# Autodesk Inventor assembly: reducer_leg
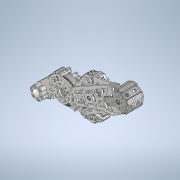
[picture p0: Inventor's stored thumbnail of the model, 180x180]
Saved by Autodesk Inventor 2020 (Build 240168000, 168)
## iProperties
Created: 2020-07-04
Part Number: reducer_leg
Document SubType Name: Assembly
Designer: psrobotics
Author: psrobotics
## Documents named in this file (26)
- D:\projects-3\biped_gen1\hardware\reducer_leg.iam
- D:\projects-3\biped_gen1\hardware\90_motor.iam
- D:\projects-3\biped_gen1\hardware\xl_20.ipt
- D:\projects-3\biped_gen1\hardware\xl_wheel_ass.iam
- D:\projects-3\biped_gen1\hardware\shell_2.ipt
- D:\projects-3\biped_gen1\hardware\shell_3.ipt
- D:\projects-3\biped_gen1\hardware\shell_4.ipt
- D:\projects-3\biped_gen1\hardware\motor_h_1.ipt
- D:\projects-3\biped_gen1\hardware\shell_5.ipt
- D:\projects-3\biped_gen1\hardware\bearing_shell_1.ipt
- D:\projects-3\biped_gen1\hardware\bearing_shell_2.ipt
- D:\projects-3\biped_gen1\hardware\xl_30_1.ipt
- D:\projects-3\biped_gen1\hardware\motor_h_4.ipt
- D:\projects-3\biped_gen1\hardware\motor_h_3_m.ipt
- D:\projects-3\biped_gen1\hardware\motor_h_5_m.ipt
- D:\projects-3\biped_gen1\hardware\bearing_35_44_5.ipt
- D:\projects-3\biped_gen1\hardware\motor_r_1.ipt
- D:\projects-3\biped_gen1\hardware\bearing_8_16_5.ipt
- D:\projects-3\biped_gen1\hardware\bearing_6_13_5.ipt
- D:\projects-3\biped_gen1\hardware\bearing_shell_3.ipt
- D:\projects-3\biped_gen1\hardware\joint_connector_1.ipt
- D:\projects-3\biped_gen1\hardware\joint_connector_2.ipt
- D:\projects-3\biped_gen1\hardware\end_holder_2.ipt
- D:\projects-3\biped_gen1\hardware\motor_h_6.ipt
- D:\projects-3\biped_gen1\hardware\end_holder_3.ipt
- D:\projects-3\biped_gen1\hardware\end_holder_4.ipt
## Components (33 placed, 25 different names)
1. 90_motor:1 [sub-assembly] — Insert:1, Insert:2, Flush:4, Insert:58, Insert:59
2. xl_20:1 — Insert:1, Insert:2, Flush:1, Tangent:1
3. xl_wheel_ass:1 [sub-assembly] — Flush:1, Tangent:1, Insert:9
4. shell_2:1 — Angle:1, Insert:9, Insert:18
5. shell_2:3 — Angle:1, Angle:2, Insert:14, Insert:17
6. shell_2:4 — Angle:2, Flush:6, Insert:15, Insert:16, Insert:33, Insert:34, Insert:81, Insert:82
7. shell_3:1 — Flush:4, Flush:5, Insert:25, Insert:26, Insert:42, Insert:43
8. shell_4:1 — Flush:5, Insert:25, Insert:26, Flush:12, Insert:40, Insert:41
9. motor_h_1:1 — Flush:6, Insert:14, Insert:15, Insert:16, Insert:17, Insert:18, Flush:10, Insert:27, Insert:28, Insert:30, Insert:31, Insert:52, Insert:53
10. shell_5:1 — Insert:35, Insert:36, Insert:37, Insert:38
11. bearing_shell_2:1 — Flush:10, Insert:27, Insert:28, Insert:75
12. xl_wheel_ass:2 [sub-assembly] — Insert:32
13. xl_30_1:1 — Insert:89
14. bearing_shell_1:1 — Insert:30, Insert:31, Insert:32
15. motor_h_4:1 — Insert:33, Insert:34, Insert:37, Insert:38, Insert:54, Insert:78, Insert:79, Flush:21, Flush:22, Flush:23, Insert:85, Insert:86, Insert:87
16. motor_h_3_m:1 — Insert:35, Insert:36, Insert:42, Insert:43, Flush:15, Insert:47, Insert:48, Insert:58, Insert:59, Flush:18, Insert:63, Insert:64, Flush:19, Insert:65, Insert:66
17. motor_h_5_m:1 — Flush:12, Insert:40, Insert:41
18. bearing_35_44_5:1 — Insert:77, Insert:87
19. motor_r_1:1 — Flush:15, Insert:47, Insert:48, Flush:17, Insert:60, Insert:61, Flush:24
20. bearing_8_16_5:1 — Insert:88, Insert:89
21. bearing_8_16_5:2 — Insert:52
22. bearing_8_16_5:3 — Insert:54
23. bearing_8_16_5:4 — Insert:53
24. bearing_6_13_5:1 — Insert:75
25. bearing_shell_3:1 — Flush:17, Insert:60, Insert:61, Insert:76
26. bearing_8_16_5:5 — Insert:76
27. joint_connector_1:1 — Flush:18, Insert:63, Insert:64
28. joint_connector_2:1 — Flush:19, Insert:65, Insert:66
29. bearing_35_44_5:2 — Insert:77, Flush:20
30. end_holder_2:1 — Insert:78, Insert:79, Flush:24, Insert:88
31. motor_h_6:1 — Flush:20, Insert:81, Insert:82, Insert:83, Insert:84
32. end_holder_3:1 — Flush:21, Flush:22, Insert:83, Insert:84
33. end_holder_4:1 — Flush:23, Insert:85, Insert:86
## Relationships (70: Insert 52, Flush 15, Angle 2, Tangent 1)
- Insert:1: 90_motor:1 ↔ xl_20:1
- Insert:2: 90_motor:1 ↔ xl_20:1
- Flush:1: xl_20:1 ↔ xl_wheel_ass:1
- Tangent:1 (1.3 mm): xl_20:1 ↔ xl_wheel_ass:1
- Angle:1 (160 deg): shell_2:1 ↔ shell_2:3
- Angle:2 (230 deg): shell_2:3 ↔ shell_2:4
- Insert:9 (-0.5 mm): xl_wheel_ass:1 ↔ shell_2:1
- Flush:4: 90_motor:1 ↔ shell_3:1
- Flush:5: shell_3:1 ↔ shell_4:1
- Flush:6: shell_2:4 ↔ motor_h_1:1
- Insert:14: shell_2:3 ↔ motor_h_1:1
- Insert:15: shell_2:4 ↔ motor_h_1:1
- Insert:16: shell_2:4 ↔ motor_h_1:1
- Insert:17: shell_2:3 ↔ motor_h_1:1
- Insert:18: shell_2:1 ↔ motor_h_1:1
- Insert:25: shell_3:1 ↔ shell_4:1
- Insert:26: shell_3:1 ↔ shell_4:1
- Flush:10: motor_h_1:1 ↔ bearing_shell_2:1
- Insert:27: motor_h_1:1 ↔ bearing_shell_2:1
- Insert:28: motor_h_1:1 ↔ bearing_shell_2:1
- Insert:30: motor_h_1:1 ↔ bearing_shell_1:1
- Insert:31: motor_h_1:1 ↔ bearing_shell_1:1
- Insert:32: xl_wheel_ass:2 ↔ bearing_shell_1:1
- Insert:33: shell_2:4 ↔ motor_h_4:1
- Insert:34: shell_2:4 ↔ motor_h_4:1
- Insert:35: shell_5:1 ↔ motor_h_3_m:1
- Insert:36: shell_5:1 ↔ motor_h_3_m:1
- Insert:37: shell_5:1 ↔ motor_h_4:1
- Insert:38: shell_5:1 ↔ motor_h_4:1
- Flush:12: shell_4:1 ↔ motor_h_5_m:1
- Insert:40: shell_4:1 ↔ motor_h_5_m:1
- Insert:41: shell_4:1 ↔ motor_h_5_m:1
- Insert:42: shell_3:1 ↔ motor_h_3_m:1
- Insert:43: shell_3:1 ↔ motor_h_3_m:1
- Flush:15: motor_h_3_m:1 ↔ motor_r_1:1
- Insert:47: motor_h_3_m:1 ↔ motor_r_1:1
- Insert:48: motor_h_3_m:1 ↔ motor_r_1:1
- Insert:52: motor_h_1:1 ↔ bearing_8_16_5:2
- Insert:53: motor_h_1:1 ↔ bearing_8_16_5:4
- Insert:54: motor_h_4:1 ↔ bearing_8_16_5:3
- Insert:58: 90_motor:1 ↔ motor_h_3_m:1
- Insert:59: 90_motor:1 ↔ motor_h_3_m:1
- Flush:17: motor_r_1:1 ↔ bearing_shell_3:1
- Insert:60: motor_r_1:1 ↔ bearing_shell_3:1
- Insert:61: motor_r_1:1 ↔ bearing_shell_3:1
- Flush:18: motor_h_3_m:1 ↔ joint_connector_1:1
- Insert:63: motor_h_3_m:1 ↔ joint_connector_1:1
- Insert:64: motor_h_3_m:1 ↔ joint_connector_1:1
- Flush:19: motor_h_3_m:1 ↔ joint_connector_2:1
- Insert:65: motor_h_3_m:1 ↔ joint_connector_2:1
- Insert:66: motor_h_3_m:1 ↔ joint_connector_2:1
- Insert:75: bearing_shell_2:1 ↔ bearing_6_13_5:1
- Insert:76: bearing_shell_3:1 ↔ bearing_8_16_5:5
- Insert:77 (26.5 mm): bearing_35_44_5:1 ↔ bearing_35_44_5:2
- Insert:78: motor_h_4:1 ↔ end_holder_2:1
- Insert:79: motor_h_4:1 ↔ end_holder_2:1
- Flush:20: bearing_35_44_5:2 ↔ motor_h_6:1
- Insert:81: shell_2:4 ↔ motor_h_6:1
- Insert:82: shell_2:4 ↔ motor_h_6:1
- Flush:21: motor_h_4:1 ↔ end_holder_3:1
- Flush:22: motor_h_4:1 ↔ end_holder_3:1
- Insert:83: motor_h_6:1 ↔ end_holder_3:1
- Insert:84: motor_h_6:1 ↔ end_holder_3:1
- Flush:23: motor_h_4:1 ↔ end_holder_4:1
- Insert:85: motor_h_4:1 ↔ end_holder_4:1
- Insert:86: motor_h_4:1 ↔ end_holder_4:1
- Flush:24: motor_r_1:1 ↔ end_holder_2:1
- Insert:87: motor_h_4:1 ↔ bearing_35_44_5:1
- Insert:88: bearing_8_16_5:1 ↔ end_holder_2:1
- Insert:89: xl_30_1:1 ↔ bearing_8_16_5:1
